# Autodesk Inventor assembly: 자동 스위치
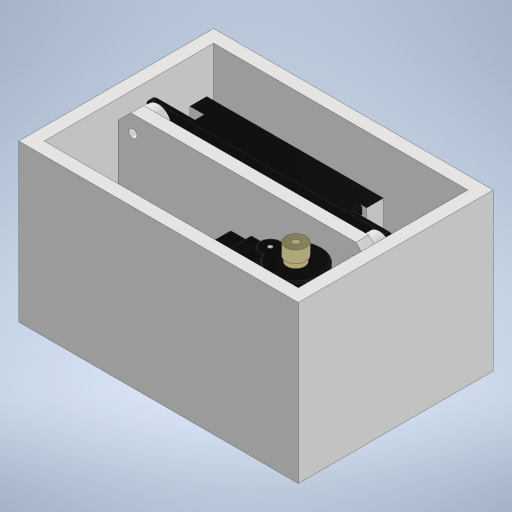
[picture p0: Inventor's stored thumbnail of the model, 512x512]
Saved by Autodesk Inventor 2023 (Build 270158000, 158)
## iProperties
Created: 2022-08-25
Part Number: 자동 스위치
Document SubType Name: Assembly
Designer: user
Author: user
## Documents named in this file (5)
- C:\Users\user\Desktop\PAI\IOT부품\자동 스위치\자동 스위치.iam
- C:\Users\user\Desktop\PAI\IOT부품\자동 스위치\esp커버.ipt
- C:\Users\user\Desktop\PAI\IOT부품\자동 스위치\전체 하우징.ipt
- C:\Users\user\Desktop\PAI\IOT부품\esp32f.ipt
- C:\Users\user\Desktop\PAI\PAI설계\범용 부품\180도 서보모터.ipt
## Components (4 placed, 4 different names)
1. esp커버:1 — 삽입:5, 삽입:6, 삽입:7
2. 전체 하우징:1 — 삽입:7, 삽입:8, 삽입:9
3. esp32f:1 — 삽입:5, 삽입:6
4. 180도 서보모터:1 — 삽입:8, 삽입:9
## Relationships (5: Insert 5)
- 삽입:5 [Insert]: esp커버:1 ↔ esp32f:1
- 삽입:6 [Insert]: esp커버:1 ↔ esp32f:1
- 삽입:7 [Insert]: esp커버:1 ↔ 전체 하우징:1
- 삽입:8 [Insert]: 전체 하우징:1 ↔ 180도 서보모터:1
- 삽입:9 [Insert]: 전체 하우징:1 ↔ 180도 서보모터:1
